# Autodesk Inventor assembly: outer
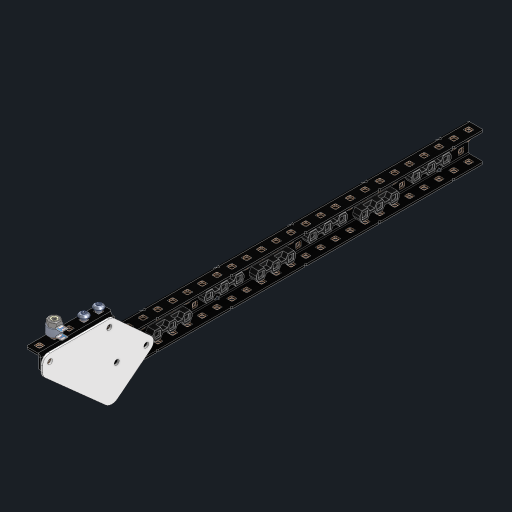
[picture p0: Inventor's stored thumbnail of the model, 512x512]
Saved by Autodesk Inventor 2024 (Build 280153000, 153)
## iProperties
Created: 2024-03-08
Part Number: outer
Document SubType Name: Assembly
Designer: Averey Ku
Author: Averey Ku
## Documents named in this file (15)
- D:\vex_robotics\hardware\cad\eca\chassis\drivebay\outer.iam
- D:\vex_robotics\hardware\cad\VEX-CAD-Inventor-1.41\Structure\C Channel\Aluminum 1x2x1\Alu C 1x2x1x27.ipt
- D:\vex_robotics\hardware\cad\VEX-CAD-Inventor-1.41\Motion\Shaft LS\Bearing Flat Low Profile.ipt
- D:\vex_robotics\hardware\cad\VEX-CAD-Inventor-1.41\Structure\Standoff\Standoff .875.ipt
- D:\vex_robotics\hardware\cad\VEX-CAD-Inventor-1.41\Structure\Standoff.ipt
- D:\vex_robotics\hardware\cad\eca\custom_parts\chassis\drivebay\sled.ipt
- D:\vex_robotics\hardware\cad\VEX-CAD-Inventor-1.41\Structure\Angle\Aluminum 1x1\Alu Angle 1x1x5.ipt
- D:\vex_robotics\hardware\cad\hardware\.375 OD Aluminum Spacer 0.875.ipt
- D:\vex_robotics\hardware\cad\VEX-CAD-Inventor-1.41\Structure\Hardware\Nut Keps.ipt
- D:\vex_robotics\hardware\cad\VEX-CAD-Inventor-1.41\Structure\Hardware\Screw Steel - Star\SScrew Star Smooth 1.250.ipt
- D:\vex_robotics\hardware\cad\VEX-CAD-Inventor-1.41\Structure\Hardware\Screw Steel - Star.ipt
- D:\vex_robotics\hardware\cad\VEX-CAD-Inventor-1.41\Structure\Hardware\Screw Shoulder Robosource.ipt
- D:\vex_robotics\hardware\cad\VEX-CAD-Inventor-1.41\Motion\Shaft LS\Shaft Collar ipts\Shaft Collar No Screw.ipt
- D:\vex_robotics\hardware\cad\VEX-CAD-Inventor-1.41\Structure\Hardware\Nut Thin Nylock.ipt
- D:\vex_robotics\hardware\cad\VEX-CAD-Inventor-1.41\Structure\Hardware\Screw Shoulder Robosource\SScrew Shoulder Smooth .500 x .18.ipt
## Components (21 placed, 11 different names)
1. Alu C 1x2x1x27:1 — Insert:1, Mate:1, Insert:2, Mate:2, Insert:3, Mate:3, Insert:4, Mate:4, Insert:5, Mate:5, Insert:6, Mate:6, Insert:7, Mate:7, Insert:8, Insert:9, Insert:12, Insert:13, Insert:14, Insert:15, Insert:16
2. Bearing Flat Low Profile:1 — Insert:1, Mate:1
3. Bearing Flat Low Profile:2 — Insert:4, Mate:4
4. Bearing Flat Low Profile:3 — Insert:2, Mate:2
5. Bearing Flat Low Profile:4 — Insert:3, Mate:3
6. Bearing Flat Low Profile:5 — Insert:5, Mate:5
7. Bearing Flat Low Profile:6 — Insert:6, Mate:6
8. Bearing Flat Low Profile:7 — Insert:7, Mate:7
9. Standoff .875:1 — Insert:8, Mate:8
10. Standoff .875:2 — Insert:9, Insert:10
11. sled:1 — Insert:11, Mate:9
12. Alu Angle 1x1x5:1 — Insert:10, Mate:8, Insert:11, Mate:9, Insert:19, Insert:21, Insert:22
13. .375 OD Aluminum Spacer 0.875:1 — Insert:12
14. Nut Keps:1 — Insert:14
15. Nut Keps:2 — Insert:13
16. SScrew Star Smooth 1.250:1 — Insert:15
17. SScrew Star Smooth 1.250:2 — Insert:16
18. Shaft Collar No Screw:1 — Insert:19, Insert:20
19. Nut Thin Nylock:1 — Insert:20
20. SScrew Shoulder Smooth .500 x .18:1 — Insert:21
21. SScrew Shoulder Smooth .500 x .18:2 — Insert:22
## Relationships (29: Insert 20, Mate 9)
- Insert:1: Alu C 1x2x1x27:1 ↔ Bearing Flat Low Profile:1
- Mate:1: Alu C 1x2x1x27:1 ↔ Bearing Flat Low Profile:1
- Insert:2: Alu C 1x2x1x27:1 ↔ Bearing Flat Low Profile:3
- Mate:2: Alu C 1x2x1x27:1 ↔ Bearing Flat Low Profile:3
- Insert:3: Alu C 1x2x1x27:1 ↔ Bearing Flat Low Profile:4
- Mate:3: Alu C 1x2x1x27:1 ↔ Bearing Flat Low Profile:4
- Insert:4: Alu C 1x2x1x27:1 ↔ Bearing Flat Low Profile:2
- Mate:4: Alu C 1x2x1x27:1 ↔ Bearing Flat Low Profile:2
- Insert:5: Alu C 1x2x1x27:1 ↔ Bearing Flat Low Profile:5
- Mate:5: Alu C 1x2x1x27:1 ↔ Bearing Flat Low Profile:5
- Insert:6: Alu C 1x2x1x27:1 ↔ Bearing Flat Low Profile:6
- Mate:6: Alu C 1x2x1x27:1 ↔ Bearing Flat Low Profile:6
- Insert:7: Alu C 1x2x1x27:1 ↔ Bearing Flat Low Profile:7
- Mate:7: Alu C 1x2x1x27:1 ↔ Bearing Flat Low Profile:7
- Insert:8: Alu C 1x2x1x27:1 ↔ Standoff .875:1
- Insert:9: Alu C 1x2x1x27:1 ↔ Standoff .875:2
- Insert:10: Standoff .875:2 ↔ Alu Angle 1x1x5:1
- Mate:8: Standoff .875:1 ↔ Alu Angle 1x1x5:1
- Insert:11: sled:1 ↔ Alu Angle 1x1x5:1
- Mate:9: sled:1 ↔ Alu Angle 1x1x5:1
- Insert:12: Alu C 1x2x1x27:1 ↔ .375 OD Aluminum Spacer 0.875:1
- Insert:13: Alu C 1x2x1x27:1 ↔ Nut Keps:2
- Insert:14: Alu C 1x2x1x27:1 ↔ Nut Keps:1
- Insert:15: Alu C 1x2x1x27:1 ↔ SScrew Star Smooth 1.250:1
- Insert:16: Alu C 1x2x1x27:1 ↔ SScrew Star Smooth 1.250:2
- Insert:19 (3.175 mm): Alu Angle 1x1x5:1 ↔ Shaft Collar No Screw:1
- Insert:20: Shaft Collar No Screw:1 ↔ Nut Thin Nylock:1
- Insert:21 (3.175 mm): Alu Angle 1x1x5:1 ↔ SScrew Shoulder Smooth .500 x .18:1
- Insert:22 (3.175 mm): Alu Angle 1x1x5:1 ↔ SScrew Shoulder Smooth .500 x .18:2
